# Autodesk Inventor assembly: sestava tělo estonsko s plechem
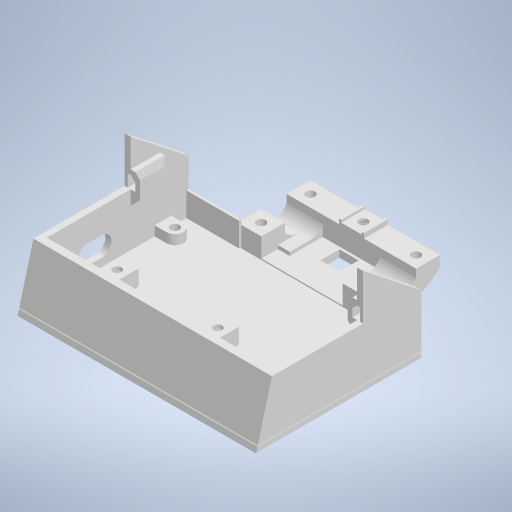
[picture p0: Inventor's stored thumbnail of the model, 512x512]
Saved by Autodesk Inventor 2024 (Build 280153000, 153)
## iProperties
Created: 2023-11-06
Part Number: sestava tělo estonsko s plechem
Document SubType Name: Assembly
Designer: jaryj
Author: jaryj
## Documents named in this file (3)
- C:\Users\jaryj\Desktop\Škola\Mini sumo\RoboCop\- 3D -\wip\Tělo s plechem\sestava tělo estonsko s plechem.iam
- C:\Users\jaryj\Desktop\Škola\Mini sumo\RoboCop\- 3D -\wip\Tělo s plechem\Plech.ipt
- C:\Users\jaryj\Desktop\Škola\Mini sumo\RoboCop\- 3D -\wip\Tělo s plechem\tělo estonsko s plechem.ipt
## Components (2 placed, 2 different names)
1. Plech:1 — Rotační:1
2. tělo estonsko s plechem:1 — Rotační:1
## Relationships (1: RevoluteJoint 1)
- Rotační:1 [RevoluteJoint]: Plech:1 ↔ tělo estonsko s plechem:1
